# Autodesk Inventor assembly: DoubleCross_Rturn_testasm
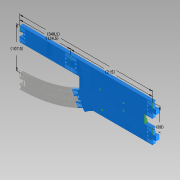
[picture p0: Inventor's stored thumbnail of the model, 180x180]
Saved by Autodesk Inventor 2021 (Build 250183000, 183)
## iProperties
Created: 2021-03-02
Part Number: DoubleCross_Rturn_testasm
Document SubType Name: Assembly
Designer: kumagai
Author: kumagai
## Documents named in this file (6)
- X:\Develop\CAD\PlaRails\DoubleCross\DoubleCross_Rturn_testasm.iam
- X:\Develop\CAD\PlaRails\DoubleCross\DoubleCross_Rturn_C.ipt
- X:\Develop\CAD\PlaRails\CurveRail\CurveRail.ipt
- X:\Develop\CAD\PlaRails\StraightRail\StraightRail_i.iam
- X:\Develop\CAD\PlaRails\StraightRail\StraightRail_i\StraightMF134.iam
- X:\Develop\CAD\PlaRails\CurveRail\CurveRail\CurveRail-342-25.ipt
## Components (3 placed, 3 different names)
1. DoubleCross_Rturn_C:1 — フラッシュ:1, フラッシュ:2, フラッシュ:3, メイト:1, メイト:2, メイト:3
2. CurveRail-342-25:1 — フラッシュ:1, メイト:2, メイト:3
3. StraightMF134:1 [sub-assembly] — フラッシュ:2, フラッシュ:3, メイト:1
## Relationships (6: Flush 3, Mate 3)
- フラッシュ:1 [Flush]: DoubleCross_Rturn_C:1 ↔ CurveRail-342-25:1
- フラッシュ:2 [Flush]: DoubleCross_Rturn_C:1 ↔ StraightMF134:1
- フラッシュ:3 [Flush]: DoubleCross_Rturn_C:1 ↔ StraightMF134:1
- メイト:1 [Mate]: DoubleCross_Rturn_C:1 ↔ StraightMF134:1
- メイト:2 [Mate]: DoubleCross_Rturn_C:1 ↔ CurveRail-342-25:1
- メイト:3 [Mate]: DoubleCross_Rturn_C:1 ↔ CurveRail-342-25:1
